# Autodesk Inventor assembly: ROBOT_ARM
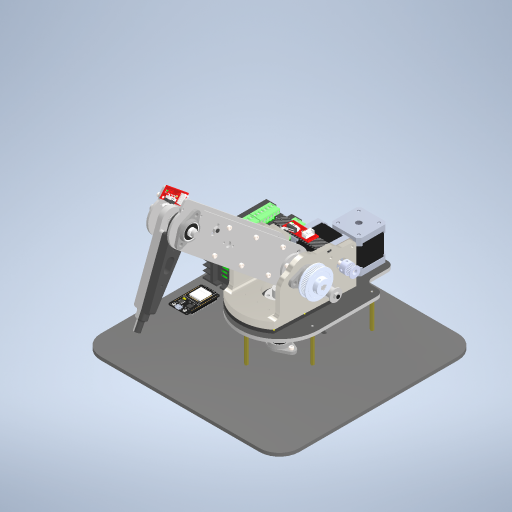
[picture p0: Inventor's stored thumbnail of the model, 512x512]
Saved by Autodesk Inventor 2023 (Build 270158000, 158)
## iProperties
Created: 2023-09-09
Part Number: ROBOT_ARM
Document SubType Name: Assembly
Designer: philo
Author: philo
## Documents named in this file (5)
- D:\02_3D_design_new\ROBOT_ARM.iam
- D:\02_3D_design_new\Base.iam
- D:\02_3D_design_new\Link2.iam
- D:\02_3D_design_new\Dexoay.iam
- D:\02_3D_design_new\Link3ver2.iam
## Components (4 placed, 4 different names)
1. Base:1 [sub-assembly] — Mate:1, Flush:1
2. Link2:1 [sub-assembly] — Mate:2, Mate:3, Mate:4, Mate:5
3. Dexoay:1 [sub-assembly] — Mate:1, Flush:1, Mate:2, Mate:3
4. Link3ver2:1 [sub-assembly] — Mate:4, Mate:5
## Relationships (6: Mate 5, Flush 1)
- Mate:1: Base:1 ↔ Dexoay:1
- Flush:1: Base:1 ↔ Dexoay:1
- Mate:2: Link2:1 ↔ Dexoay:1
- Mate:3 (15 mm): Link2:1 ↔ Dexoay:1
- Mate:4: Link2:1 ↔ Link3ver2:1
- Mate:5 (3 mm): Link2:1 ↔ Link3ver2:1
